# Autodesk Inventor assembly: TZS 1270 top funnel
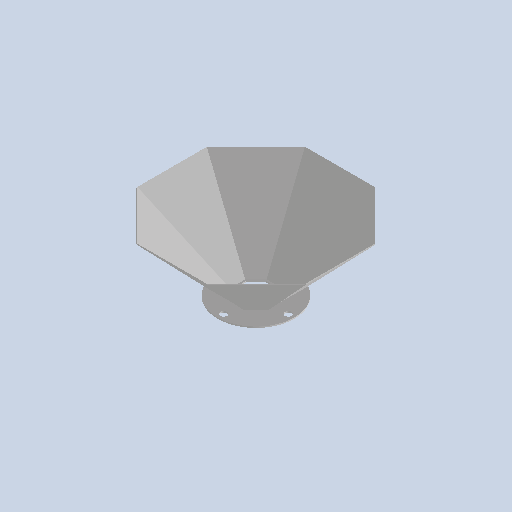
[picture p0: Inventor's stored thumbnail of the model, 512x512]
Saved by Autodesk Inventor 2025 (Build 290162010, 162A)
## iProperties
Created: 2025-07-11
Part Number: TZS 1270 top funnel
Document SubType Name: Assembly
Designer: user
Author: user
## Documents named in this file (3)
- C:\Users\pokla\Documents\Inventor\TZS-Tazovskiy\Фильтр D1200\TZS 1270 top funnel.iam
- C:\Users\pokla\Documents\Inventor\TZS-Tazovskiy\Фильтр D1200\TZS 1271 top funnel wall.ipt
- C:\Users\pokla\Documents\Inventor\TZS-Tazovskiy\Фильтр D1200\TZS 1272 funnel FLANGE 50-90.ipt
## Components (3 placed, 2 different names)
1. TZS 1272 funnel FLANGE 50-90.ipt:1 — Mate:1, Mate:2, Mate:3, Mate:4, Mate:6, Mate:7
2. TZS 1271 top funnel wall.ipt:1 — Mate:1, Mate:2, Mate:5, Mate:7
3. TZS 1271 top funnel wall.ipt:2 — Mate:3, Mate:4, Mate:5, Mate:6
## Relationships (7: Mate 7)
- Mate:1: TZS 1272 funnel FLANGE 50-90.ipt:1 ↔ TZS 1271 top funnel wall.ipt:1
- Mate:2: TZS 1272 funnel FLANGE 50-90.ipt:1 ↔ TZS 1271 top funnel wall.ipt:1
- Mate:3: TZS 1272 funnel FLANGE 50-90.ipt:1 ↔ TZS 1271 top funnel wall.ipt:2
- Mate:4: TZS 1272 funnel FLANGE 50-90.ipt:1 ↔ TZS 1271 top funnel wall.ipt:2
- Mate:5: TZS 1271 top funnel wall.ipt:1 ↔ TZS 1271 top funnel wall.ipt:2
- Mate:6 (-2.87 mm): TZS 1272 funnel FLANGE 50-90.ipt:1 ↔ TZS 1271 top funnel wall.ipt:2
- Mate:7 (-2.87 mm): TZS 1272 funnel FLANGE 50-90.ipt:1 ↔ TZS 1271 top funnel wall.ipt:1
